# Autodesk Inventor assembly: Container and stand
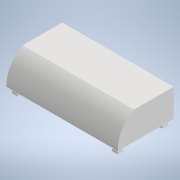
[picture p0: Inventor's stored thumbnail of the model, 180x180]
Saved by Autodesk Inventor 2020 (Build 240168000, 168)
## iProperties
Created: 2021-05-03
Part Number: Container and stand
Document SubType Name: Assembly
Designer: chick
Author: chick
## Documents named in this file (3)
- C:\Users\chick\Desktop\Deisng Project CAD\Container and stand.iam
- C:\Users\chick\Desktop\Deisng Project CAD\Container.ipt
- C:\Users\chick\Desktop\Deisng Project CAD\Stand.ipt
## Components (5 placed, 2 different names)
1. Container:1 — Mate:1, Mate:2, Mate:3, Mate:4, Mate:5, Mate:6, Mate:7, Mate:8
2. Stand:1 — Mate:1, Mate:2
3. Stand:2 — Mate:3, Mate:4
4. Stand:3 — Mate:7, Mate:8
5. Stand:4 — Mate:5, Mate:6
## Relationships (8: Mate 8)
- Mate:1: Container:1 ↔ Stand:1
- Mate:2: Container:1 ↔ Stand:1
- Mate:3: Container:1 ↔ Stand:2
- Mate:4: Container:1 ↔ Stand:2
- Mate:5: Container:1 ↔ Stand:4
- Mate:6: Container:1 ↔ Stand:4
- Mate:7: Container:1 ↔ Stand:3
- Mate:8: Container:1 ↔ Stand:3
